# Autodesk Inventor assembly: optotether_v03
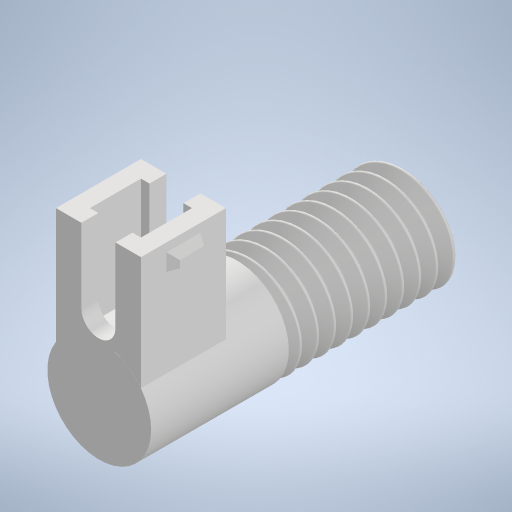
[picture p0: Inventor's stored thumbnail of the model, 512x512]
Saved by Autodesk Inventor 2023 (Build 270158000, 158)
## iProperties
Created: 2024-05-14
Part Number: optotether_v03
Document SubType Name: Assembly
Designer: Akramilab
Author: Akramilab
## Documents named in this file (3)
- C:\Projects\Inventor\OptoTetherSpring\optotether_v03.iam
- C:\Projects\Inventor\tetherspring_screw\SCREW_nogap.ipt
- C:\Projects\Inventor\OptoTetherSpring\snapfit_part_v02.ipt
## Components (2 placed, 2 different names)
1. snapfit_part_v02:1
2. SCREW_nogap:1
## Relationships (1: Flush 1)
- [Flush]: snapfit_part_v02:1 ↔ SCREW_nogap:1
